# Autodesk Inventor assembly: Upper_bearing_support_inside_print
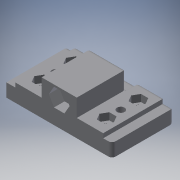
[picture p0: Inventor's stored thumbnail of the model, 180x180]
Saved by Autodesk Inventor 2019.3 (Build 233278000, 278)
## iProperties
Created: 2020-09-10
Part Number: Upper_bearing_support_inside_print
Material: Generisch
Document SubType Name: Assembly
Designer: Nicolas Frick
Author: Nicolas Frick
## Documents named in this file (2)
- C:\Users\Nicolas Frick\Sync\OneDrive\airhockeybot\mechanical_design\common_cad_parts\print_models\upper\Upper_bearing_support_inside_print.iam
- C:\Users\Nicolas Frick\Sync\OneDrive\airhockeybot\mechanical_design\inventor\Upper_bearing_support_inside.ipt
## Components (1 placed, 1 different names)
1. Upper_bearing_support_inside:1 — Passend:1, Passend:2, Passend:3
## Relationships (3: Mate 3)
- Passend:1 [Mate]: Upper_bearing_support_inside:1
- Passend:2 [Mate]: Upper_bearing_support_inside:1
- Passend:3 [Mate]: Upper_bearing_support_inside:1
